# Autodesk Inventor assembly: SPM
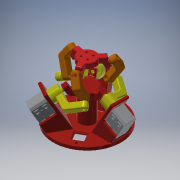
[picture p0: Inventor's stored thumbnail of the model, 180x180]
Saved by Autodesk Inventor 2019 (Build 230136000, 136)
## iProperties
Created: 2022-08-22
Part Number: SPM
Document SubType Name: Assembly
Designer: zreik
Author: zreik
## Documents named in this file (6)
- D:\Documents\HIAST\4th year\4th Year Project\Design\Current\SPM.iam
- D:\Documents\HIAST\4th year\4th Year Project\Design\Current\BottomPlatform.ipt
- D:\Documents\HIAST\4th year\4th Year Project\Design\Current\TopPlatform.ipt
- D:\Documents\HIAST\4th year\4th Year Project\Design\Current\Link1.ipt
- D:\Documents\HIAST\4th year\4th Year Project\Design\Current\Link2.ipt
- D:\Documents\HIAST\4th year\4th Year Project\Design\Current\XL-320.ipt
## Components (11 placed, 5 different names)
1. BottomPlatform:1 — Flush:1, Flush:2, Flush:3, Mate:1, Mate:2, Mate:3, Angle:1, Mate:12, Mate:15, Mate:18, Mate:21, Mate:22, Mate:23
2. TopPlatform:1 — Mate:4, Mate:5, Mate:6, Angle:1, Mate:14, Mate:17, Mate:19
3. Link1:1 — Mate:12, Mate:13
4. Link2:1 — Mate:13, Mate:14
5. Link1:2 — Mate:15, Mate:16
6. Link2:2 — Mate:16, Mate:17
7. Link1:3 — Mate:18, Mate:20
8. Link2:3 — Mate:19, Mate:20
9. XL-320:1 — Mate:21, Mate:22, Mate:23
10. XL-320:2
11. XL-320:3
## Component patterns: (3 elements, first: XL-320:1)
## Relationships (27: Mate 23, Flush 3, Angle 1)
- Flush:1: BottomPlatform:1
- Flush:2: BottomPlatform:1
- Flush:3: BottomPlatform:1
- Mate:1: BottomPlatform:1
- Mate:2: BottomPlatform:1
- Mate:3: BottomPlatform:1
- Mate:4: TopPlatform:1
- Mate:5: TopPlatform:1
- Mate:6: TopPlatform:1
- Mate:7
- Mate:8
- Mate:9
- Mate:10
- Mate:11
- Angle:1 (0 deg): BottomPlatform:1 ↔ TopPlatform:1
- Mate:12: BottomPlatform:1 ↔ Link1:1
- Mate:13: Link1:1 ↔ Link2:1
- Mate:14: TopPlatform:1 ↔ Link2:1
- Mate:15: BottomPlatform:1 ↔ Link1:2
- Mate:16: Link1:2 ↔ Link2:2
- Mate:17: TopPlatform:1 ↔ Link2:2
- Mate:18: BottomPlatform:1 ↔ Link1:3
- Mate:19: TopPlatform:1 ↔ Link2:3
- Mate:20: Link1:3 ↔ Link2:3
- Mate:21: BottomPlatform:1 ↔ XL-320:1
- Mate:22: BottomPlatform:1 ↔ XL-320:1
- Mate:23: BottomPlatform:1 ↔ XL-320:1
